# Autodesk Inventor assembly: Assembly base2
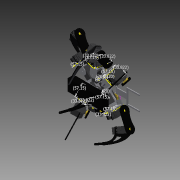
[picture p0: Inventor's stored thumbnail of the model, 180x180]
Saved by Autodesk Inventor 2015 (Build 190159000, 159)
## iProperties
Created: 2015-12-27
Part Number: Assembly base2
Document SubType Name: Assembly
Designer: William
Author: William
## Documents named in this file (17)
- E:\Data William\Robotik\berkaki1\FIXED\Assembly base2.iam
- E:\Data William\Robotik\berkaki1\BASE NEWWWW3.ipt
- E:\Data William\Robotik\berkaki1\servo.ipt
- E:\Data William\Robotik\berkaki1\Assembly2.1.iam
- E:\Data William\Robotik\berkaki1\Assembly2.iam
- E:\Data William\Robotik\berkaki1\tibia servo.iam
- E:\Data William\Robotik\berkaki1\femurpendek horn.iam
- E:\Data William\Robotik\berkaki1\tibia servo2.iam
- E:\Data William\Robotik\berkaki1\bayi.ipt
- E:\Data William\Robotik\ROBUSTA\Part1.ipt
- E:\Data William\Robotik\ROBUSTA\Baterai.ipt
- E:\Data William\Robotik\ROBUSTA\Spacer 2cm.ipt
- E:\Data William\Robotik\ROBUSTA\Spacer 1cm.ipt
- E:\Data William\Robotik\ROBUSTA\Bearing Besar.ipt
- E:\Data William\Robotik\berkaki1\braket dan horn.iam
- C:\Users\William\Documents\Inventor\Content Center Files\R2015\en-US\DIN 7985 (H)\DIN 7985 (H) - M2.5x14-H.ipt
- C:\Users\William\Documents\Inventor\Content Center Files\R2015\en-US\ISO 4036(1)\ISO 4036 - M2.5(1).ipt
## Components (44 placed, 16 different names)
1. BASE NEWWWW3:1 — Mate:55, Mate:56, Mate:58, Mate:70, Mate:71, Mate:85, Mate:86, Mate:87, Mate:88, Mate:90
2. servo:1 — Mate:115, Mate:116
3. servo:2 — Mate:94, Mate:103
4. servo:3 — Mate:107, Mate:108
5. servo:4 — Mate:55, Mate:56, Mate:111, Mate:112
6. servo:5 — Mate:58, Mate:109, Mate:110
7. servo:6 — Mate:113, Mate:114
8. Assembly2.1:1 [sub-assembly] — Mate:76, Mate:77, Mate:119, Mate:120
9. Assembly2.1:2 [sub-assembly] — Mate:73, Mate:74, Mate:117, Mate:118
10. Assembly2.1:3 [sub-assembly] — Mate:35, Mate:36, Mate:127, Mate:128, Mate:129
11. Assembly2:1 [sub-assembly] — Mate:41, Mate:42, Mate:125, Mate:126
12. Assembly2:2 [sub-assembly] — Mate:80, Mate:81, Mate:123, Mate:124
13. Assembly2:3 [sub-assembly] — Mate:78, Mate:79, Mate:121, Mate:122
14. tibia servo:1 [sub-assembly] — Mate:43, Mate:44
15. tibia servo:2 [sub-assembly] — Mate:45, Mate:46
16. tibia servo:3 [sub-assembly] — Mate:47, Mate:48
17. femurpendek horn:1 [sub-assembly] — Mate:53, Mate:54, Mate:76, Mate:77
18. femurpendek horn:2 [sub-assembly] — Mate:72, Mate:73, Mate:74, Mate:75
19. femurpendek horn:3 [sub-assembly] — Mate:35, Mate:36, Mate:49, Mate:50
20. femurpendek horn:4 [sub-assembly] — Mate:43, Mate:44, Mate:78, Mate:79
21. femurpendek horn:5 [sub-assembly] — Mate:45, Mate:46, Mate:80, Mate:81
22. femurpendek horn:6 [sub-assembly] — Mate:41, Mate:42, Mate:47, Mate:48
23. tibia servo2:1 [sub-assembly] — Mate:49, Mate:50
24. tibia servo2:2 [sub-assembly] — Mate:72, Mate:75
25. tibia servo2:3 [sub-assembly] — Mate:53, Mate:54
26. bayi:1 — Mate:70, Mate:71
27. Baterai:1
28. Spacer 2cm:1 — Mate:85, Mate:86
29. Spacer 2cm:2 — Mate:87, Mate:88
30. Spacer 2cm:3 — Mate:90, Mate:91, Mate:92
31. Spacer 1cm:1 — Mate:91, Mate:92, Mate:93
32. Part1:1 — Mate:93, Mate:101, Mate:105
33. braket dan horn:1 [sub-assembly] — Mate:94, Insert:1, Mate:97, Mate:103, Mate:119, Mate:120
34. DIN 7985 (H) M2.5x14-H:1 — Insert:1, Mate:96, Mate:99, Mate:100, Mate:104
35. DIN EN 24036 M2.5:1 — Mate:96, Mate:97
36. Bearing Besar:2 — Mate:99, Mate:102, Insert:2
37. Bearing Besar:3 — Mate:100, Mate:101, Mate:102
38. DIN EN 24036 M2.5:2 — Mate:104, Mate:105
39. DIN EN 24036 M2.5:3 — Insert:2
40. braket dan horn:3 [sub-assembly] — Mate:107, Mate:108, Mate:117, Mate:118
41. braket dan horn:4 [sub-assembly] — Mate:111, Mate:112, Mate:127, Mate:128, Mate:129
42. braket dan horn:5 [sub-assembly] — Mate:113, Mate:114, Mate:123, Mate:124
43. braket dan horn:6 [sub-assembly] — Mate:109, Mate:110, Mate:125, Mate:126
44. braket dan horn:7 [sub-assembly] — Mate:115, Mate:116, Mate:121, Mate:122
## Relationships (72: Mate 70, Insert 2)
- Mate:35: Assembly2.1:3 ↔ femurpendek horn:3
- Mate:36: Assembly2.1:3 ↔ femurpendek horn:3
- Mate:41: Assembly2:1 ↔ femurpendek horn:6
- Mate:42: Assembly2:1 ↔ femurpendek horn:6
- Mate:43: tibia servo:1 ↔ femurpendek horn:4
- Mate:44: tibia servo:1 ↔ femurpendek horn:4
- Mate:45: tibia servo:2 ↔ femurpendek horn:5
- Mate:46: tibia servo:2 ↔ femurpendek horn:5
- Mate:47: tibia servo:3 ↔ femurpendek horn:6
- Mate:48: tibia servo:3 ↔ femurpendek horn:6
- Mate:49: femurpendek horn:3 ↔ tibia servo2:1
- Mate:50: femurpendek horn:3 ↔ tibia servo2:1
- Mate:53: femurpendek horn:1 ↔ tibia servo2:3
- Mate:54: femurpendek horn:1 ↔ tibia servo2:3
- Mate:55: BASE NEWWWW3:1 ↔ servo:4
- Mate:56: BASE NEWWWW3:1 ↔ servo:4
- Mate:58: BASE NEWWWW3:1 ↔ servo:5
- Mate:70: BASE NEWWWW3:1 ↔ bayi:1
- Mate:71: BASE NEWWWW3:1 ↔ bayi:1
- Mate:72: femurpendek horn:2 ↔ tibia servo2:2
- Mate:73: Assembly2.1:2 ↔ femurpendek horn:2
- Mate:74: Assembly2.1:2 ↔ femurpendek horn:2
- Mate:75: femurpendek horn:2 ↔ tibia servo2:2
- Mate:76: Assembly2.1:1 ↔ femurpendek horn:1
- Mate:77: Assembly2.1:1 ↔ femurpendek horn:1
- Mate:78: Assembly2:3 ↔ femurpendek horn:4
- Mate:79: Assembly2:3 ↔ femurpendek horn:4
- Mate:80: Assembly2:2 ↔ femurpendek horn:5
- Mate:81: Assembly2:2 ↔ femurpendek horn:5
- Mate:85: BASE NEWWWW3:1 ↔ Spacer 2cm:1
- Mate:86: BASE NEWWWW3:1 ↔ Spacer 2cm:1
- Mate:87: BASE NEWWWW3:1 ↔ Spacer 2cm:2
- Mate:88: BASE NEWWWW3:1 ↔ Spacer 2cm:2
- Mate:90: BASE NEWWWW3:1 ↔ Spacer 2cm:3
- Mate:91: Spacer 2cm:3 ↔ Spacer 1cm:1
- Mate:92: Spacer 2cm:3 ↔ Spacer 1cm:1
- Mate:93: Spacer 1cm:1 ↔ Part1:1
- Mate:94: servo:2 ↔ braket dan horn:1
- Insert:1: braket dan horn:1 ↔ DIN 7985 (H) M2.5x14-H:1
- Mate:96: DIN 7985 (H) M2.5x14-H:1 ↔ DIN EN 24036 M2.5:1
- Mate:97: braket dan horn:1 ↔ DIN EN 24036 M2.5:1
- Mate:99: DIN 7985 (H) M2.5x14-H:1 ↔ Bearing Besar:2
- Mate:100: DIN 7985 (H) M2.5x14-H:1 ↔ Bearing Besar:3
- Mate:101: Part1:1 ↔ Bearing Besar:3
- Mate:102: Bearing Besar:2 ↔ Bearing Besar:3
- Mate:103: servo:2 ↔ braket dan horn:1
- Mate:104: DIN 7985 (H) M2.5x14-H:1 ↔ DIN EN 24036 M2.5:2
- Mate:105: Part1:1 ↔ DIN EN 24036 M2.5:2
- Insert:2: Bearing Besar:2 ↔ DIN EN 24036 M2.5:3
- Mate:107: servo:3 ↔ braket dan horn:3
- Mate:108: servo:3 ↔ braket dan horn:3
- Mate:109: servo:5 ↔ braket dan horn:6
- Mate:110: servo:5 ↔ braket dan horn:6
- Mate:111: servo:4 ↔ braket dan horn:4
- Mate:112: servo:4 ↔ braket dan horn:4
- Mate:113: servo:6 ↔ braket dan horn:5
- Mate:114: servo:6 ↔ braket dan horn:5
- Mate:115: servo:1 ↔ braket dan horn:7
- Mate:116: servo:1 ↔ braket dan horn:7
- Mate:117: Assembly2.1:2 ↔ braket dan horn:3
- Mate:118: Assembly2.1:2 ↔ braket dan horn:3
- Mate:119: Assembly2.1:1 ↔ braket dan horn:1
- Mate:120: Assembly2.1:1 ↔ braket dan horn:1
- Mate:121: Assembly2:3 ↔ braket dan horn:7
- Mate:122: Assembly2:3 ↔ braket dan horn:7
- Mate:123: Assembly2:2 ↔ braket dan horn:5
- Mate:124: Assembly2:2 ↔ braket dan horn:5
- Mate:125: Assembly2:1 ↔ braket dan horn:6
- Mate:126: Assembly2:1 ↔ braket dan horn:6
- Mate:127: Assembly2.1:3 ↔ braket dan horn:4
- Mate:128: Assembly2.1:3 ↔ braket dan horn:4
- Mate:129: Assembly2.1:3 ↔ braket dan horn:4
